# Autodesk Inventor assembly: LowerBody_MIR
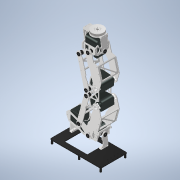
[picture p0: Inventor's stored thumbnail of the model, 180x180]
Saved by Autodesk Inventor 2020 (Build 240168000, 168)
## iProperties
Created: 2016-08-23
Part Number: LowerBody_MIR
Material: 一般
Document SubType Name: Assembly
Designer: Masato
Mass: 952.391 g
Surface Area: 2598.56 cm^2
Volume: 454.704 cm^3
Density: 2.09453 g/cm^3
Author: hiro
## Documents named in this file (12)
- C:\Users\naoki\Documents\Inventor\CitBrains\git_clone\OpenPlatform167\0915\OpenPlatform_ver3_0\LowerBody_MIR.iam
- C:\Users\naoki\Documents\Inventor\CitBrains\git_clone\OpenPlatform167\0915\OpenPlatform_ver3_0\LowerBody\Leg_joint_roll\Leg_Joint_roll.iam
- C:\Users\naoki\Documents\Inventor\CitBrains\git_clone\OpenPlatform167\0915\OpenPlatform_ver3_0\LowerBody\Slider_crank\Slider_crank_mechanism.iam
- C:\Users\naoki\Documents\Inventor\CitBrains\git_clone\OpenPlatform167\0915\OpenPlatform_ver3_0\LowerBody\Leg_joit\Leg_joint.iam
- C:\Users\naoki\Documents\Inventor\CitBrains\git_clone\OpenPlatform167\0915\OpenPlatform_ver3_0\LowerBody\Link\UpperFrontLink.iam
- C:\Users\naoki\Documents\Inventor\CitBrains\git_clone\OpenPlatform167\0915\OpenPlatform_ver3_0\LowerBody\Link\UpperBackLink.iam
- C:\Users\naoki\Documents\Inventor\CitBrains\git_clone\OpenPlatform167\0915\OpenPlatform_ver3_0\LowerBody\Knee\Knee.iam
- C:\Users\naoki\Documents\Inventor\CitBrains\git_clone\OpenPlatform167\0915\OpenPlatform_ver3_0\LowerBody\Link\LowerFrontLink.iam
- C:\Users\naoki\Documents\Inventor\CitBrains\git_clone\OpenPlatform167\0915\OpenPlatform_ver3_0\LowerBody\Link\LowerBackLink.iam
- C:\Users\naoki\Documents\Inventor\CitBrains\git_clone\OpenPlatform167\0915\OpenPlatform_ver3_0\LowerBody\Ankle\Ankle.iam
- C:\Users\naoki\Documents\Inventor\CitBrains\git_clone\OpenPlatform167\0915\OpenPlatform_ver3_0\LowerBody\Ankle\Ankle_side_pitch.iam
- C:\Users\naoki\Documents\Inventor\CitBrains\git_clone\OpenPlatform167\0915\OpenPlatform_ver3_0\LowerBody\Foot\Foot_MIR.iam
## Components (12 placed, 11 different names)
1. 付け根ロール_1:1 [sub-assembly] — フラッシュ:26, フラッシュ:25, メイト:23, 挿入:97, 角度:4, 角度:12, 角度:4, 挿入:20
2. Slider_crank_mechanism:1 [sub-assembly] — 挿入:97, 挿入:109
3. 付け根_1:1 [sub-assembly] — 挿入:109, 角度:4, 挿入:19, 挿入:20, 挿入:21
4. UpperFrontLink:1 [sub-assembly] — 角度:12, 挿入:111, 挿入:21
5. UpperBackLink:1 [sub-assembly] — 挿入:19, 挿入:22
6. 膝_1:1 [sub-assembly] — 挿入:98, 挿入:111, 挿入:22, 挿入:23
7. LowerFrontLink:1 [sub-assembly] — 挿入:98, 挿入:29, 角度:5
8. LowerBackLink:1 [sub-assembly] — 挿入:23, 挿入:27, 挿入:28
9. 足首_1:1 [sub-assembly] — 挿入:24, 挿入:25, 挿入:30, 挿入:31
10. 足首_独立ピッチ_1:1 [sub-assembly] — 挿入:25, 挿入:28, 挿入:29
11. 足首_独立ピッチ_1:2 [sub-assembly] — 挿入:24, 挿入:27
12. Foot_MIR:1 [sub-assembly] — 角度:4, 挿入:30, 挿入:31, 角度:5
## Relationships (23: Insert 16, Angle 4, Mate 2, Flush 1)
- フラッシュ:26 [Flush]: 付け根ロール_1:1
- フラッシュ:25 [Mate]: 付け根ロール_1:1
- メイト:23 [Mate]: 付け根ロール_1:1
- 挿入:97 [Insert]: 付け根ロール_1:1 ↔ Slider_crank_mechanism:1
- 挿入:98 [Insert]: 膝_1:1 ↔ LowerFrontLink:1
- 挿入:109 [Insert]: Slider_crank_mechanism:1 ↔ 付け根_1:1
- 角度:4 [Angle] (0 deg): 付け根ロール_1:1 ↔ 付け根_1:1
- 角度:12 [Angle] (-15 deg): 付け根ロール_1:1 ↔ UpperFrontLink:1
- 挿入:111 [Insert]: UpperFrontLink:1 ↔ 膝_1:1
- 角度:4 [Angle] (0 deg): 付け根ロール_1:1 ↔ Foot_MIR:1
- 挿入:19 [Insert]: 付け根_1:1 ↔ UpperBackLink:1
- 挿入:20 [Insert]: 付け根ロール_1:1 ↔ 付け根_1:1
- 挿入:21 [Insert]: 付け根_1:1 ↔ UpperFrontLink:1
- 挿入:22 [Insert]: UpperBackLink:1 ↔ 膝_1:1
- 挿入:23 [Insert]: 膝_1:1 ↔ LowerBackLink:1
- 挿入:24 [Insert]: 足首_1:1 ↔ 足首_独立ピッチ_1:2
- 挿入:25 [Insert]: 足首_1:1 ↔ 足首_独立ピッチ_1:1
- 挿入:27 [Insert]: LowerBackLink:1 ↔ 足首_独立ピッチ_1:2
- 挿入:28 [Insert]: LowerBackLink:1 ↔ 足首_独立ピッチ_1:1
- 挿入:29 [Insert]: LowerFrontLink:1 ↔ 足首_独立ピッチ_1:1
- 挿入:30 [Insert]: 足首_1:1 ↔ Foot_MIR:1
- 挿入:31 [Insert]: 足首_1:1 ↔ Foot_MIR:1
- 角度:5 [Angle] (-15 deg): LowerFrontLink:1 ↔ Foot_MIR:1
